# Autodesk Inventor assembly: Tip_support
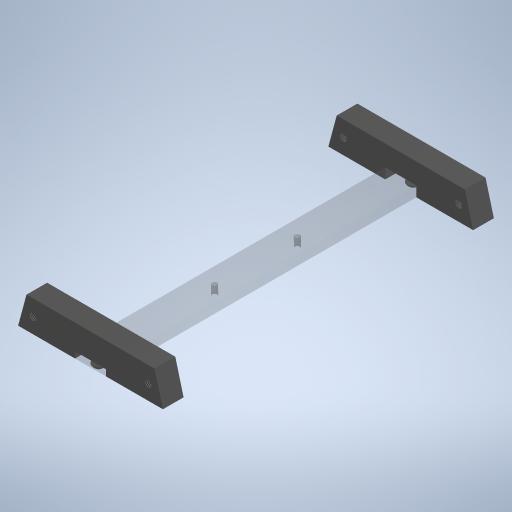
[picture p0: Inventor's stored thumbnail of the model, 512x512]
Saved by Autodesk Inventor 2023 (Build 270158000, 158)
## iProperties
Created: 2023-03-29
Part Number: Tip_support
Document SubType Name: Assembly
Designer: ASARe-DAQ-PC
Author: ASARe-DAQ-PC
## Documents named in this file (4)
- D:\EB camera\model of EB camera\for manufacture\Tip_support.iam
- D:\EB camera\model of EB camera\for manufacture\Tip_support_1.ipt
- D:\EB camera\model of EB camera\for manufacture\Tip_support_2.ipt
- D:\EB camera\model of EB camera\for manufacture\Screw M3 Hex 8mm.ipt
## Components (5 placed, 3 different names)
1. Tip_support_1:1 — Mate:4, Mate:5, Flush:1
2. Tip_support_1:2 — Mate:1, Mate:2, Mate:3
3. Tip_support_2:1 — Mate:1, Mate:2, Mate:3, Mate:4, Mate:5, Flush:1, Insert:1, Insert:2
4. Screw M3 Hex 8mm:5 — Insert:2
5. Screw M3 Hex 8mm:6 — Insert:1
## Relationships (8: Mate 5, Insert 2, Flush 1)
- Mate:1: Tip_support_1:2 ↔ Tip_support_2:1
- Mate:2: Tip_support_1:2 ↔ Tip_support_2:1
- Mate:3: Tip_support_1:2 ↔ Tip_support_2:1
- Mate:4: Tip_support_1:1 ↔ Tip_support_2:1
- Mate:5: Tip_support_1:1 ↔ Tip_support_2:1
- Flush:1: Tip_support_1:1 ↔ Tip_support_2:1
- Insert:1: Tip_support_2:1 ↔ Screw M3 Hex 8mm:6
- Insert:2: Tip_support_2:1 ↔ Screw M3 Hex 8mm:5
